# Autodesk Inventor assembly: roue_roulements
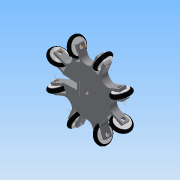
[picture p0: Inventor's stored thumbnail of the model, 180x180]
Saved by Autodesk Inventor 2015 (Build 190159000, 159)
## iProperties
Created: 2016-03-31
Part Number: roue_roulements
Document SubType Name: Assembly
Designer: Gregwar
Author: Gregwar
## Documents named in this file (3)
- C:\Users\Gregwar\Desktop\laser\omni\roue_roulements.iam
- C:\Users\Gregwar\Desktop\laser\omni\roue.ipt
- C:\Users\Gregwar\Desktop\laser\omni\roulement_joint.ipt
## Components (9 placed, 2 different names)
1. roue:1 — Placage:1, Placage:2
2. roulement_joint:1 — Placage:1, Placage:2
3. roulement_joint:2
4. roulement_joint:3
5. roulement_joint:4
6. roulement_joint:5
7. roulement_joint:6
8. roulement_joint:7
9. roulement_joint:8
## Component patterns: (8 elements, first: roulement_joint:1)
## Relationships (2: Mate 2)
- Placage:1 [Mate]: roue:1 ↔ roulement_joint:1
- Placage:2 [Mate]: roue:1 ↔ roulement_joint:1
